# Autodesk Inventor assembly: Сборка1
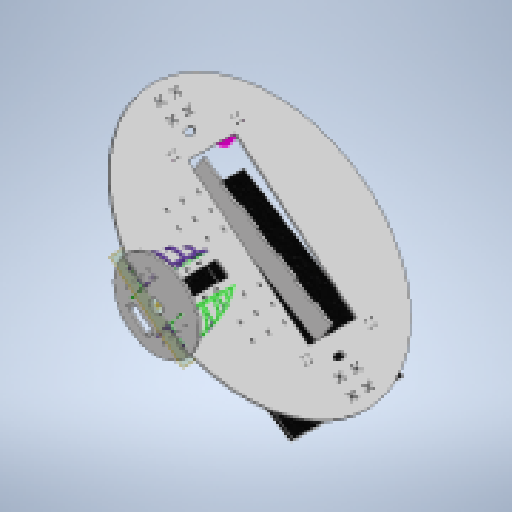
[picture p0: Inventor's stored thumbnail of the model, 512x512]
Saved by Autodesk Inventor 2023.1 (Build 271208000, 208)
## iProperties
Created: 2025-02-03
Part Number: Сборка1
Document SubType Name: Assembly
Designer: baranovaem
Author: baranovaem
## Documents named in this file (10)
- C:\Users\DELL\reposGitHub\Cheburashka\Cheburashka_construction\face\лицо\Сборка1.iam
- C:\Users\DELL\reposGitHub\Cheburashka\Cheburashka_construction\face\лицо\лицо1.ipt
- C:\Users\DELL\reposGitHub\Cheburashka\Cheburashka_construction\face\лицо\магнит_стойка.ipt
- C:\Users\DELL\reposGitHub\Cheburashka\Cheburashka_construction\face\лицо\монитор.ipt
- C:\Users\baranovaem\Downloads\экс\стенка.ipt
- C:\Users\DELL\reposGitHub\Cheburashka\Cheburashka_construction\face\лицо\основа_лица.ipt
- C:\Users\DELL\reposGitHub\Cheburashka\Cheburashka_construction\face\лицо\парус1.ipt
- C:\Users\DELL\reposGitHub\Cheburashka\Cheburashka_construction\face\лицо\стенкаB.ipt
- C:\Users\DELL\reposGitHub\Cheburashka\Cheburashka_construction\face\лицо\парус2.ipt
- \\sch239.net\UserHomes\Students\other\baranovaem\cheburashka\Cheburashka-main\Cheburashka_construction\platform\4ad8d019baf454c6bbd45c2c6ffb6783.ipt
## Components (17 placed, 9 different names)
1. лицо1:1 — Совмещение:1, Совмещение:2, Угол:1, Совмещение:68, Совмещение:69, Совмещение:70, Совмещение:72, Совмещение:73, Совмещение:74, Совмещение:76, Совмещение:78, Совмещение:79, Совмещение:82, Совмещение:84, Совмещение:85, Совмещение:86
2. магнит_стойка:1 — Совмещение:90
3. магнит_стойка:2 — Совмещение:88, Совмещение:91, Совмещение:92
4. магнит_стойка:3 — Совмещение:87
5. магнит_стойка:4 — Совмещение:89
6. монитор:1 — Совмещение:91, Совмещение:92
7. стенка:1
8. основа_лица:1 — Совмещение:71, Совмещение:72, Совмещение:75, Совмещение:77, Совмещение:80, Совмещение:87, Совмещение:88, Совмещение:89, Совмещение:90
9. парус1:2 — Совмещение:68
10. парус1:4 — Совмещение:69, Совмещение:70
11. стенкаB:1
12. парус2:1
13. парус2:2
14. 4ad8d019baf454c6bbd45c2c6ffb6783:1 — Совмещение:71, Совмещение:73, Совмещение:84
15. 4ad8d019baf454c6bbd45c2c6ffb6783:2 — Совмещение:74, Совмещение:75, Совмещение:76, Совмещение:85
16. 4ad8d019baf454c6bbd45c2c6ffb6783:3 — Совмещение:77, Совмещение:78, Совмещение:82
17. 4ad8d019baf454c6bbd45c2c6ffb6783:4 — Совмещение:79, Совмещение:80, Совмещение:86
## Relationships (26: Mate 25, Angle 1)
- Совмещение:1 [Mate]: лицо1:1
- Совмещение:2 [Mate]: лицо1:1
- Угол:1 [Angle] (0 deg): лицо1:1
- Совмещение:68 [Mate]: лицо1:1 ↔ парус1:2
- Совмещение:69 [Mate]: лицо1:1 ↔ парус1:4
- Совмещение:70 [Mate]: лицо1:1 ↔ парус1:4
- Совмещение:71 [Mate]: основа_лица:1 ↔ 4ad8d019baf454c6bbd45c2c6ffb6783:1
- Совмещение:72 [Mate]: лицо1:1 ↔ основа_лица:1
- Совмещение:73 [Mate]: лицо1:1 ↔ 4ad8d019baf454c6bbd45c2c6ffb6783:1
- Совмещение:74 [Mate]: лицо1:1 ↔ 4ad8d019baf454c6bbd45c2c6ffb6783:2
- Совмещение:75 [Mate]: основа_лица:1 ↔ 4ad8d019baf454c6bbd45c2c6ffb6783:2
- Совмещение:76 [Mate]: лицо1:1 ↔ 4ad8d019baf454c6bbd45c2c6ffb6783:2
- Совмещение:77 [Mate]: основа_лица:1 ↔ 4ad8d019baf454c6bbd45c2c6ffb6783:3
- Совмещение:78 [Mate]: лицо1:1 ↔ 4ad8d019baf454c6bbd45c2c6ffb6783:3
- Совмещение:79 [Mate]: лицо1:1 ↔ 4ad8d019baf454c6bbd45c2c6ffb6783:4
- Совмещение:80 [Mate]: основа_лица:1 ↔ 4ad8d019baf454c6bbd45c2c6ffb6783:4
- Совмещение:82 [Mate]: лицо1:1 ↔ 4ad8d019baf454c6bbd45c2c6ffb6783:3
- Совмещение:84 [Mate]: лицо1:1 ↔ 4ad8d019baf454c6bbd45c2c6ffb6783:1
- Совмещение:85 [Mate]: лицо1:1 ↔ 4ad8d019baf454c6bbd45c2c6ffb6783:2
- Совмещение:86 [Mate]: лицо1:1 ↔ 4ad8d019baf454c6bbd45c2c6ffb6783:4
- Совмещение:87 [Mate]: магнит_стойка:3 ↔ основа_лица:1
- Совмещение:88 [Mate]: магнит_стойка:2 ↔ основа_лица:1
- Совмещение:89 [Mate]: магнит_стойка:4 ↔ основа_лица:1
- Совмещение:90 [Mate]: магнит_стойка:1 ↔ основа_лица:1
- Совмещение:91 [Mate]: магнит_стойка:2 ↔ монитор:1
- Совмещение:92 [Mate]: магнит_стойка:2 ↔ монитор:1
